# Autodesk Inventor assembly: IR SENSOR ASSMBLY
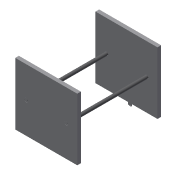
[picture p0: Inventor's stored thumbnail of the model, 180x180]
Saved by Autodesk Inventor 2019 (Build 230136000, 136)
## iProperties
Created: 2019-10-10
Part Number: IR SENSOR ASSMBLY
Document SubType Name: Assembly
Designer: Admin
Author: Admin
## Documents named in this file (4)
- C:\Users\Admin\Documents\IR SENSOR ASSMBLY.iam
- C:\Users\Admin\Documents\top support.ipt
- C:\Users\Admin\Documents\23CM NUT.ipt
- C:\Users\Admin\Documents\ir sensor.ipt
## Components (8 placed, 3 different names)
1. top support:1 — Mate:1, Insert:3, Rotational:1
2. top support:2 — Mate:2, Mate:3, Mate:4, Insert:1, Mate:5, Insert:2, Angle:1, Mate:6, Rigid:1, Mate:7, Mate:8
3. 23CM NUT:1 — Mate:1, Mate:2, Mate:5, Insert:2, Insert:3, Rotational:1
4. 23CM NUT:2 — Mate:3, Mate:4, Insert:1
5. ir sensor:1 — Angle:1, Mate:6
6. ir sensor:3
7. ir sensor:4
8. ir sensor:5 — Rigid:1, Mate:7, Mate:8
## Relationships (14: Mate 8, Insert 3, RevoluteJoint 1, Angle 1, WeldJoint 1)
- Mate:1: top support:1 ↔ 23CM NUT:1
- Mate:2: top support:2 ↔ 23CM NUT:1
- Mate:3: top support:2 ↔ 23CM NUT:2
- Mate:4: top support:2 ↔ 23CM NUT:2
- Insert:1: top support:2 ↔ 23CM NUT:2
- Mate:5: top support:2 ↔ 23CM NUT:1
- Insert:2: top support:2 ↔ 23CM NUT:1
- Insert:3: top support:1 ↔ 23CM NUT:1
- Rotational:1 [RevoluteJoint]: top support:1 ↔ 23CM NUT:1
- Angle:1 (0 deg): top support:2 ↔ ir sensor:1
- Mate:6: top support:2 ↔ ir sensor:1
- Rigid:1 [WeldJoint]: top support:2 ↔ ir sensor:5
- Mate:7: top support:2 ↔ ir sensor:5
- Mate:8: top support:2 ↔ ir sensor:5
